# Autodesk Inventor assembly: Piece_I
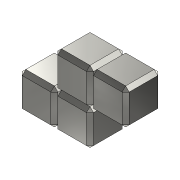
[picture p0: Inventor's stored thumbnail of the model, 180x180]
Saved by Autodesk Inventor 2021 (Build 250183000, 183)
## iProperties
Created: 2021-04-01
Part Number: Piece_I
Document SubType Name: Assembly
Designer: Tran Duc Viet
Mass: 4958.27 g
Surface Area: 526.693 cm^2
Volume: 472.667 cm^3
Density: 10.49 g/cm^3
Author: Tran Duc Viet
## Documents named in this file (2)
- C:\Users\davei\Desktop\School\Léto 2020-2021\VRM\Projects\P2\Piece_I.iam
- C:\Users\davei\Desktop\School\Léto 2020-2021\VRM\Projects\P2\ElementaryCube_SILVER.ipt
## Components (4 placed, 1 different names)
1. ElementaryCube_SILVER:1 — Mate:1, Flush:1, Flush:2
2. ElementaryCube_SILVER:2 — Mate:1, Flush:1, Flush:2, Flush:3, Mate:4, Flush:7
3. ElementaryCube_SILVER:3 — Flush:3, Mate:3, Flush:5, Flush:6, Mate:4, Flush:7
4. ElementaryCube_SILVER:4 — Mate:3, Flush:5, Flush:6
## Relationships (9: Flush 6, Mate 3)
- Mate:1: ElementaryCube_SILVER:1 ↔ ElementaryCube_SILVER:2
- Flush:1: ElementaryCube_SILVER:1 ↔ ElementaryCube_SILVER:2
- Flush:2: ElementaryCube_SILVER:1 ↔ ElementaryCube_SILVER:2
- Flush:3: ElementaryCube_SILVER:2 ↔ ElementaryCube_SILVER:3
- Mate:3: ElementaryCube_SILVER:3 ↔ ElementaryCube_SILVER:4
- Flush:5: ElementaryCube_SILVER:3 ↔ ElementaryCube_SILVER:4
- Flush:6: ElementaryCube_SILVER:3 ↔ ElementaryCube_SILVER:4
- Mate:4: ElementaryCube_SILVER:2 ↔ ElementaryCube_SILVER:3
- Flush:7: ElementaryCube_SILVER:2 ↔ ElementaryCube_SILVER:3
